# Autodesk Inventor assembly: Flex Cable Assembly V1
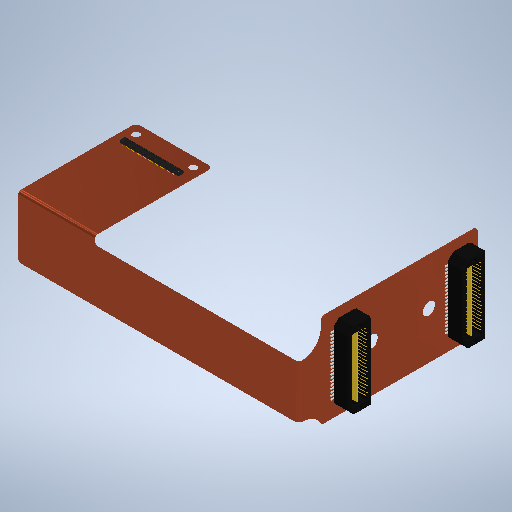
[picture p0: Inventor's stored thumbnail of the model, 512x512]
Saved by Autodesk Inventor 2025 (Build 290162000, 162)
## iProperties
Created: 2024-08-05
Part Number: Flex Cable Assembly V1
Document SubType Name: Assembly
Designer: Caleb Fangmeier
Author: Caleb Fangmeier
## Documents named in this file (4)
- C:\Users\cfang\Desktop\nebraska-silicon-lab\Hardware\ETL\Module Assembly\Tamale Assembly Plate FLEX V1\Flex Cable Assembly V1.iam
- C:\Users\cfang\Desktop\nebraska-silicon-lab\Hardware\ETL\Module Assembly\Tamale Assembly Plate FLEX V1\105897078002\105897078002.ipt
- C:\Users\cfang\Desktop\nebraska-silicon-lab\Hardware\ETL\Module Assembly\Tamale Assembly Plate FLEX V1\Flex V1.ipt
- C:\Users\cfang\Desktop\nebraska-silicon-lab\Hardware\ETL\Module Assembly\Tamale Assembly Plate FLEX V1\QTE-020\QTE-020-01-L-D.iam
## Components (4 placed, 3 different names)
1. Flex V1:1 — Mate:1, Mate:2, Mate:3, Flush:1, Flush:4, Flush:5, Flush:6
2. Kyocera 5897 — Mate:1, Flush:5, Flush:6
3. QTE-020-01-L-D:1 [sub-assembly] — Mate:2, Flush:1, Flush:2, Flush:3
4. QTE-020-01-L-D:2 [sub-assembly] — Mate:3, Flush:2, Flush:3, Flush:4
## Relationships (9: Flush 6, Mate 3)
- Mate:1: Flex V1:1 ↔ Kyocera 5897
- Mate:2: Flex V1:1 ↔ QTE-020-01-L-D:1
- Mate:3: Flex V1:1 ↔ QTE-020-01-L-D:2
- Flush:1 (2.25 mm): Flex V1:1 ↔ QTE-020-01-L-D:1
- Flush:2 (30 mm): QTE-020-01-L-D:1 ↔ QTE-020-01-L-D:2
- Flush:3: QTE-020-01-L-D:1 ↔ QTE-020-01-L-D:2
- Flush:4 (2.25 mm): Flex V1:1 ↔ QTE-020-01-L-D:2
- Flush:5 (5.176 mm): Flex V1:1 ↔ Kyocera 5897
- Flush:6 (2.255 mm): Flex V1:1 ↔ Kyocera 5897
